# Autodesk Inventor assembly: 組合1
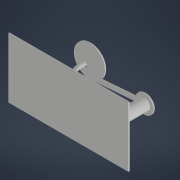
[picture p0: Inventor's stored thumbnail of the model, 180x180]
Saved by Autodesk Inventor 2021 (Build 250183000, 183)
## iProperties
Created: 2020-12-30
Part Number: 組合1
Document SubType Name: Assembly
Designer: zihon
Author: zihon
## Documents named in this file (8)
- C:\Users\zihon\Desktop\New folder\組合1.iam
- C:\Users\zihon\Desktop\New folder\架.ipt
- C:\Users\zihon\Desktop\New folder\零件1.ipt
- C:\Users\zihon\Desktop\New folder\零件2.ipt
- C:\Users\zihon\Desktop\New folder\零件3.ipt
- C:\Users\zihon\Desktop\New folder\零件4.ipt
- C:\Users\zihon\Desktop\New folder\軸.ipt
- C:\Users\zihon\Desktop\New folder\螺旋.ipt
## Components (7 placed, 7 different names)
1. 架:1 — 貼合:2, 齊平:1, 貼合:4, 貼合:8, 貼合:9, 貼合:11, 貼合:15, 貼合:16, 貼合:18, 貼合:27, 貼合:28, 貼合:29, 齊平:3, 齊平:4, 齊平:5, 貼合:30, 貼合:31
2. 零件1:1 — 貼合:4, 相切:1, 貼合:18
3. 零件2:1 — 貼合:27, 貼合:28, 相切:5
4. 零件3:1 — 貼合:8, 相切:3, 貼合:16
5. 零件4:1 — 貼合:9, 相切:4, 貼合:15
6. 軸:1 — 貼合:11, 相切:1, 相切:3, 相切:4, 相切:5, 貼合:31
7. 螺旋:1 — 貼合:20, 貼合:29, 齊平:3
## Relationships (22: Mate 14, Flush 4, Tangent 4)
- 貼合:2 [Mate]: 架:1
- 齊平:1 [Flush]: 架:1
- 貼合:4 [Mate]: 架:1 ↔ 零件1:1
- 貼合:8 [Mate]: 架:1 ↔ 零件3:1
- 貼合:9 [Mate]: 架:1 ↔ 零件4:1
- 貼合:11 [Mate]: 架:1 ↔ 軸:1
- 相切:1 [Tangent]: 零件1:1 ↔ 軸:1
- 相切:3 [Tangent]: 零件3:1 ↔ 軸:1
- 相切:4 [Tangent]: 零件4:1 ↔ 軸:1
- 貼合:15 [Mate]: 架:1 ↔ 零件4:1
- 貼合:16 [Mate]: 架:1 ↔ 零件3:1
- 貼合:18 [Mate]: 架:1 ↔ 零件1:1
- 貼合:20 [Mate]: 螺旋:1
- 貼合:27 [Mate]: 架:1 ↔ 零件2:1
- 貼合:28 [Mate]: 架:1 ↔ 零件2:1
- 相切:5 [Tangent]: 零件2:1 ↔ 軸:1
- 貼合:29 [Mate]: 架:1 ↔ 螺旋:1
- 齊平:3 [Flush]: 架:1 ↔ 螺旋:1
- 齊平:4 [Flush]: 架:1
- 齊平:5 [Flush]: 架:1
- 貼合:30 [Mate]: 架:1
- 貼合:31 [Mate]: 架:1 ↔ 軸:1
